# Autodesk Inventor assembly: pcb_stackup
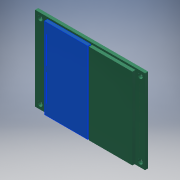
[picture p0: Inventor's stored thumbnail of the model, 180x180]
Saved by Autodesk Inventor 2019.4 (Build 234330000, 330)
## iProperties
Created: 2021-01-22
Part Number: pcb_stackup
Document SubType Name: Assembly
Designer: caleb
Author: caleb
## Documents named in this file (3)
- C:\Users\cfang\Desktop\nebraska-silicon-lab\CAD\ETL\Module Assembly\Mock Assembly\pcb_stackup.iam
- C:\Users\cfang\Desktop\nebraska-silicon-lab\CAD\ETL\Module Assembly\Mock Assembly\etroc.iam
- C:\Users\cfang\Desktop\nebraska-silicon-lab\CAD\ETL\Module Assembly\Mock Assembly\base.iam
## Components (3 placed, 2 different names)
1. etroc:1 [sub-assembly] — Mate:1, Angle:1, Flush:1
2. base:1 [sub-assembly] — Mate:1, Angle:1, Mate:2, Angle:2
3. etroc:2 [sub-assembly] — Mate:2, Angle:2, Flush:1
## Relationships (5: Mate 2, Angle 2, Flush 1)
- Mate:1: etroc:1 ↔ base:1
- Angle:1 (0 deg): etroc:1 ↔ base:1
- Mate:2: base:1 ↔ etroc:2
- Angle:2 (0 deg): base:1 ↔ etroc:2
- Flush:1: etroc:1 ↔ etroc:2
